# Autodesk Inventor assembly: Giant-Snes-Gamepad
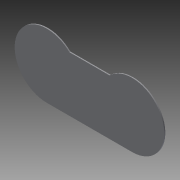
[picture p0: Inventor's stored thumbnail of the model, 180x180]
Saved by Autodesk Inventor 2014 SP1 (Build 180222100, 222)
## iProperties
Created: 2014-01-12
Part Number: Giant-Snes-Gamepad
Document SubType Name: Assembly
Designer: tuleu
Author: tuleu
## Documents named in this file (3)
- C:\Users\tuleu\Documents\giant-snes-gamepad\cad\Giant-Snes-Gamepad.iam
- C:\Users\tuleu\Documents\giant-snes-gamepad\cad\Base_Left.ipt
- C:\Users\tuleu\Documents\giant-snes-gamepad\cad\Base_Right.ipt
## Components (2 placed, 2 different names)
1. Base_Left:1 — Mate:1, Flush:1, Flush:2, Mate:2
2. Base_Right:1 — Mate:1, Flush:1, Flush:2
## Relationships (4: Mate 2, Flush 2)
- Mate:1: Base_Left:1 ↔ Base_Right:1
- Flush:1: Base_Left:1 ↔ Base_Right:1
- Flush:2: Base_Left:1 ↔ Base_Right:1
- Mate:2: Base_Left:1
